# Autodesk Inventor assembly: Claw
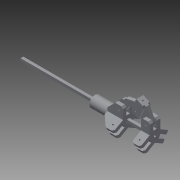
[picture p0: Inventor's stored thumbnail of the model, 180x180]
Saved by Autodesk Inventor 2014 SP1 (Build 180222100, 222)
## iProperties
Created: 2014-01-26
Part Number: Claw
Document SubType Name: Assembly
Designer: tom
Author: tom
## Documents named in this file (6)
- C:\Users\tom\Documents\GitHub\Boat_Bot\Inventor\Claw.iam
- C:\Users\tom\Documents\GitHub\Boat_Bot\Inventor\Coupler.ipt
- C:\Users\tom\Documents\GitHub\Boat_Bot\Inventor\Plunger2.ipt
- C:\Users\tom\Documents\GitHub\Boat_Bot\Inventor\Finger Joint.ipt
- C:\Users\tom\Documents\GitHub\Boat_Bot\Inventor\linkage.ipt
- C:\Users\tom\Documents\GitHub\Boat_Bot\Inventor\Push Rod.ipt
## Components (9 placed, 6 different names)
1. Coupler:1
2. Plunger2:1
3. Push Rod:1
4. Finger:1
5. linkage:1
6. Finger Joint:2
7. linkage:2
8. Finger Joint:3
9. linkage:3
## Component patterns: (3 elements, first: Finger:1 + linkage:1)
## Relationships (7: RevoluteJoint 3, Mate 2, Flush 1, TranslationJoint 1)
- [RevoluteJoint]: Coupler:1 ↔ linkage:1
- [Flush]: Plunger2:1 ↔ Push Rod:1
- [Mate]: Plunger2:1 ↔ Push Rod:1
- [Mate]: Plunger2:1 ↔ Push Rod:1
- [RevoluteJoint]: Finger:1 ↔ linkage:1
- [RevoluteJoint]: Plunger2:1 ↔ Finger:1
- [TranslationJoint]: Coupler:1 ↔ Push Rod:1
## Named parameters: d0_d9 = 0 mm, d1_d10 = 20.665723 deg
